# Autodesk Inventor assembly: Intake V3
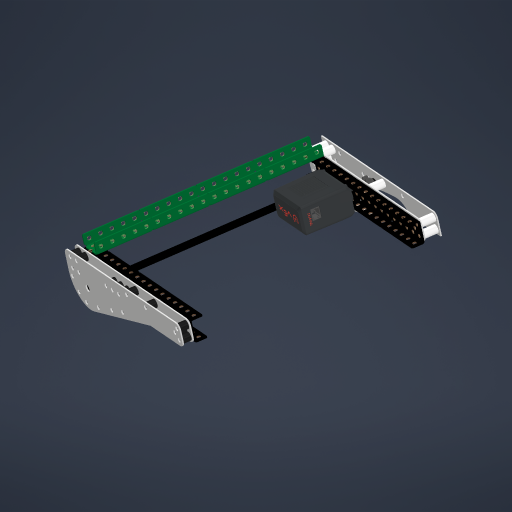
[picture p0: Inventor's stored thumbnail of the model, 512x512]
Saved by Autodesk Inventor 2023.4 (Build 274418000, 418)
## iProperties
Created: 2023-12-16
Part Number: Intake V3
Document SubType Name: Assembly
Designer: diego
Author: diego
## Documents named in this file (20)
- C:\Users\diego\OneDrive\Documents\GitHub\2024-599Z\2024-599Z\Cad\NEW Intake\plan x intake.iam
- C:\Users\diego\OneDrive\Documents\GitHub\2024-599Z\2024-599Z\Cad\Library\VEX-CAD-Inventor-1.4.0\Structure\C Channel\Aluminum 1x2x1\Alu C 1x2x1x17.ipt
- C:\Users\diego\OneDrive\Documents\GitHub\2024-599Z\2024-599Z\Cad\Library\VEX-CAD-Inventor-1.4.0\Motion\Shaft HS\HS Spacer\HSpacer .0625.ipt
- C:\Users\diego\OneDrive\Documents\GitHub\2024-599Z\2024-599Z\Cad\Library\VEX-CAD-Inventor-1.4.0\Motion\Shaft HS\Shaft HS\Shaft HS 11.0 in.ipt
- C:\Users\diego\OneDrive\Documents\GitHub\2024-599Z\2024-599Z\Cad\Library\VEX-CAD-Inventor-1.4.0\Motion\Sprockets\6P Sprocket\6P 8T Sprocket, No Insert.iam
- C:\Users\diego\OneDrive\Documents\GitHub\2024-599Z\2024-599Z\Cad\Library\VEX-CAD-Inventor-1.4.0\Motion\Shaft HS\Low Profile HS Shaft Collar.ipt
- C:\Users\diego\OneDrive\Documents\GitHub\2024-599Z\2024-599Z\Cad\Library\VEX-CAD-Inventor-1.4.0\Motion\Spacers\Spacer Nylon .313 OD\NSpacer .313 OD x .500.ipt
- C:\Users\Meer\OneDrive\Documents\GitHub\2024-599Z\Cad\Library\VEX-CAD-Inventor-1.4.0\Motion\Spacers\Spacer Nylon .313 OD.ipt
- C:\Users\diego\OneDrive\Documents\GitHub\2024-599Z\2024-599Z\Cad\Library\VEX-CAD-Inventor-1.4.0\Motion\Spacers\Spacer Nylon .313 OD\NSpacer .313 OD x .125.ipt
- C:\Users\Meer\OneDrive\Documents\GitHub\2024-599Z\Cad\Library\VEX-CAD-Inventor-1.4.0\Motion\Sprockets\6P Sprocket.iam
- C:\Users\Meer\OneDrive\Documents\GitHub\2024-599Z\Cad\Library\VEX-CAD-Inventor-1.4.0\Motion\Shaft HS\HS Spacer.ipt
- C:\Users\diego\OneDrive\Documents\GitHub\2024-599Z\2024-599Z\Cad\Library\VEX-CAD-Inventor-1.4.0\Motion\Sprockets\6P Sprocket\6P 8T Sprocket, Square.iam
- C:\Users\diego\OneDrive\Documents\GitHub\2024-599Z\2024-599Z\Cad\Library\VEX-CAD-Inventor-1.4.0\Structure\C Channel\Aluminum 1x2x1\Alu C 1x2x1x20.ipt
- C:\Users\Meer\OneDrive\Documents\GitHub\2024-599Z\Cad\Library\VEX-CAD-Inventor-1.4.0\Motion\Shaft HS\Shaft HS.ipt
- C:\Users\diego\OneDrive\Documents\GitHub\2024-599Z\2024-599Z\Cad\NEW CNC Poly\intake poly x.ipt
- C:\Users\diego\OneDrive\Documents\GitHub\2024-599Z\2024-599Z\Cad\Library\VEX-CAD-Inventor-1.4.0\Electronics\Motors with Screws\SteelM-StarS.iam
- C:\Users\Meer\OneDrive\Documents\GitHub\2024-599Z\Cad\Library\VEX-CAD-Inventor-1.4.0\Electronics\Motors with Screws.iam
- C:\Users\diego\OneDrive\Documents\GitHub\2024-599Z\2024-599Z\Cad\Poly for Evan\Intake poly cut (1)\Intake poly cut (1).ipt
- C:\Users\diego\OneDrive\Documents\GitHub\2024-599Z\2024-599Z\Cad\Library\VEX-CAD-Inventor-1.4.0\Motion\Spacers\Spacer Nylon .375 OD\NSpacer .375 OD x .375.ipt
- C:\Users\diego\OneDrive\Documents\GitHub\2024-599Z\2024-599Z\Cad\Library\VEX-CAD-Inventor-1.4.0\Motion\Spacers\Spacer Nylon .375 OD.ipt
## Components (56 placed, 13 different names)
1. Shaft HS 11.0 in:1 — Insert:227
2. Alu C 1x2x1x17:1 — Insert:138, Insert:139, Insert:146, Insert:147, Insert:208, Insert:209
3. Alu C 1x2x1x17:2 — Insert:136, Insert:137, Insert:205, Insert:206, Insert:222
4. 6P 8T Sprocket, No Insert:4 [sub-assembly] — Insert:24, Insert:39
5. HSpacer .0625:8 — Insert:24, Insert:224
6. HSpacer .0625:12 — Insert:39, Insert:225
7. NSpacer .313 OD x .500:1 — Insert:71, Insert:160
8. NSpacer .313 OD x .500:4 — Insert:72, Insert:159
9. NSpacer .313 OD x .500:6 — Insert:63, Insert:150
10. NSpacer .313 OD x .500:8 — Insert:74, Insert:157
11. NSpacer .313 OD x .500:9 — Insert:62, Insert:212
12. NSpacer .313 OD x .500:10 — Insert:61, Insert:214
13. NSpacer .313 OD x .500:12 — Insert:67, Insert:154
14. NSpacer .313 OD x .500:13 — Insert:73, Insert:158
15. NSpacer .313 OD x .500:15 — Insert:69, Insert:156
16. NSpacer .313 OD x .125:19 — Insert:61, Insert:211
17. NSpacer .313 OD x .125:20 — Insert:63
18. NSpacer .313 OD x .125:23 — Insert:62
19. NSpacer .313 OD x .125:24 — Insert:67
20. NSpacer .313 OD x .125:26 — Insert:69, Insert:213
21. NSpacer .313 OD x .125:27 — Insert:71
22. NSpacer .313 OD x .125:29 — Insert:72
23. NSpacer .313 OD x .125:30 — Insert:73
24. NSpacer .313 OD x .125:31 — Insert:74
25. NSpacer .313 OD x .500:34 — Insert:163
26. NSpacer .313 OD x .500:35 — Insert:162
27. NSpacer .313 OD x .125:47
28. NSpacer .313 OD x .125:59
29. Low Profile HS Shaft Collar:4 — Insert:223
30. HSpacer .0625:14 — Insert:135
31. HSpacer .0625:15 — Insert:134, Insert:210
32. 6P 8T Sprocket, Square:6 [sub-assembly] — Insert:134, Insert:135
33. Alu C 1x2x1x20:1 — Insert:136, Insert:137, Insert:138, Insert:139
34. intake poly x:1 — Insert:146, Insert:147, Insert:150, Insert:154, Insert:156, Insert:157, Insert:158, Insert:159, Insert:160, Insert:162, Insert:163, Insert:210, Insert:212, Insert:214, Insert:225
35. intake poly x:2 — Insert:205, Insert:206, Insert:221
36. NSpacer .375 OD x .375:12
37. NSpacer .375 OD x .375:18
38. NSpacer .375 OD x .375:4 — Insert:218
39. NSpacer .375 OD x .375:13
40. NSpacer .375 OD x .375:7 — Insert:219
41. NSpacer .375 OD x .375:5
42. NSpacer .375 OD x .375:3 — Insert:215
43. NSpacer .375 OD x .375:15
44. NSpacer .375 OD x .375:2
45. NSpacer .375 OD x .375:1 — Insert:222, Insert:226
46. NSpacer .375 OD x .375:6 — Insert:216
47. NSpacer .375 OD x .375:10
48. NSpacer .375 OD x .375:14
49. NSpacer .375 OD x .375:16
50. NSpacer .375 OD x .375:11 — Insert:221
51. NSpacer .375 OD x .375:17
52. NSpacer .375 OD x .375:9
53. NSpacer .375 OD x .375:8 — Insert:220
54. intake poly x:3 — Insert:215, Insert:216, Insert:218, Insert:219, Insert:220, Insert:226, Insert:227
55. SteelM-StarS:1 [sub-assembly] — Insert:208, Insert:209
56. Intake poly cut (1):1 — Insert:211, Insert:213, Insert:223, Insert:224
## Relationships (63: Insert 63)
- Insert:24: 6P 8T Sprocket, No Insert:4 ↔ HSpacer .0625:8
- Insert:39: 6P 8T Sprocket, No Insert:4 ↔ HSpacer .0625:12
- Insert:61: NSpacer .313 OD x .500:10 ↔ NSpacer .313 OD x .125:19
- Insert:62: NSpacer .313 OD x .500:9 ↔ NSpacer .313 OD x .125:23
- Insert:63: NSpacer .313 OD x .500:6 ↔ NSpacer .313 OD x .125:20
- Insert:67: NSpacer .313 OD x .500:12 ↔ NSpacer .313 OD x .125:24
- Insert:69: NSpacer .313 OD x .500:15 ↔ NSpacer .313 OD x .125:26
- Insert:71: NSpacer .313 OD x .500:1 ↔ NSpacer .313 OD x .125:27
- Insert:72: NSpacer .313 OD x .500:4 ↔ NSpacer .313 OD x .125:29
- Insert:73: NSpacer .313 OD x .500:13 ↔ NSpacer .313 OD x .125:30
- Insert:74: NSpacer .313 OD x .500:8 ↔ NSpacer .313 OD x .125:31
- [Insert]: NSpacer .313 OD x .500:34 ↔ NSpacer .313 OD x .125:47
- [Insert]: NSpacer .313 OD x .500:35 ↔ NSpacer .313 OD x .125:59
- Insert:134: HSpacer .0625:15 ↔ 6P 8T Sprocket, Square:6
- Insert:135: HSpacer .0625:14 ↔ 6P 8T Sprocket, Square:6
- Insert:136: Alu C 1x2x1x17:2 ↔ Alu C 1x2x1x20:1
- Insert:137: Alu C 1x2x1x17:2 ↔ Alu C 1x2x1x20:1
- Insert:138: Alu C 1x2x1x17:1 ↔ Alu C 1x2x1x20:1
- Insert:139: Alu C 1x2x1x17:1 ↔ Alu C 1x2x1x20:1
- Insert:146: Alu C 1x2x1x17:1 ↔ intake poly x:1
- Insert:147: Alu C 1x2x1x17:1 ↔ intake poly x:1
- Insert:150: NSpacer .313 OD x .500:6 ↔ intake poly x:1
- Insert:154: NSpacer .313 OD x .500:12 ↔ intake poly x:1
- Insert:156: NSpacer .313 OD x .500:15 ↔ intake poly x:1
- Insert:157: NSpacer .313 OD x .500:8 ↔ intake poly x:1
- Insert:158: NSpacer .313 OD x .500:13 ↔ intake poly x:1
- Insert:159: NSpacer .313 OD x .500:4 ↔ intake poly x:1
- Insert:160: NSpacer .313 OD x .500:1 ↔ intake poly x:1
- Insert:162: NSpacer .313 OD x .500:35 ↔ intake poly x:1
- Insert:163: NSpacer .313 OD x .500:34 ↔ intake poly x:1
- [Insert]: NSpacer .375 OD x .375:5 ↔ intake poly x:3
- [Insert]: NSpacer .375 OD x .375:10 ↔ intake poly x:3
- [Insert]: NSpacer .375 OD x .375:16 ↔ intake poly x:3
- [Insert]: NSpacer .375 OD x .375:11 ↔ intake poly x:3
- [Insert]: NSpacer .375 OD x .375:15 ↔ intake poly x:3
- [Insert]: NSpacer .375 OD x .375:14 ↔ intake poly x:3
- [Insert]: NSpacer .375 OD x .375:13 ↔ intake poly x:3
- [Insert]: NSpacer .375 OD x .375:12 ↔ intake poly x:3
- [Insert]: NSpacer .375 OD x .375:18 ↔ intake poly x:3
- [Insert]: NSpacer .375 OD x .375:9 ↔ intake poly x:3
- [Insert]: NSpacer .375 OD x .375:17 ↔ intake poly x:3
- [Insert]: NSpacer .375 OD x .375:2 ↔ intake poly x:3
- Insert:205: Alu C 1x2x1x17:2 ↔ intake poly x:2
- Insert:206: Alu C 1x2x1x17:2 ↔ intake poly x:2
- Insert:208: Alu C 1x2x1x17:1 ↔ SteelM-StarS:1
- Insert:209: Alu C 1x2x1x17:1 ↔ SteelM-StarS:1
- Insert:210: HSpacer .0625:15 ↔ intake poly x:1
- Insert:211: NSpacer .313 OD x .125:19 ↔ Intake poly cut (1):1
- Insert:212: NSpacer .313 OD x .500:9 ↔ intake poly x:1
- Insert:213: NSpacer .313 OD x .125:26 ↔ Intake poly cut (1):1
- Insert:214: NSpacer .313 OD x .500:10 ↔ intake poly x:1
- Insert:215: NSpacer .375 OD x .375:3 ↔ intake poly x:3
- Insert:216: NSpacer .375 OD x .375:6 ↔ intake poly x:3
- Insert:218: NSpacer .375 OD x .375:4 ↔ intake poly x:3
- Insert:219: NSpacer .375 OD x .375:7 ↔ intake poly x:3
- Insert:220: NSpacer .375 OD x .375:8 ↔ intake poly x:3
- Insert:221: intake poly x:2 ↔ NSpacer .375 OD x .375:11
- Insert:222: Alu C 1x2x1x17:2 ↔ NSpacer .375 OD x .375:1
- Insert:223: Low Profile HS Shaft Collar:4 ↔ Intake poly cut (1):1
- Insert:224: HSpacer .0625:8 ↔ Intake poly cut (1):1
- Insert:225: HSpacer .0625:12 ↔ intake poly x:1
- Insert:226: NSpacer .375 OD x .375:1 ↔ intake poly x:3
- Insert:227: Shaft HS 11.0 in:1 ↔ intake poly x:3
## Named parameters: d129_d111 = 0 mm, d141_d124 = 0 mm, d232_d216 = 0 mm, d236_d220 = 0 mm, d237_d221 = 0 mm, d238_d222 = 0 mm, d239_d223 = 0 mm, d240_d224 = 0 mm, d241_d225 = 0 mm, d242_d226 = 0 mm, d243_d227 = 0 mm, d244_d228 = 0 mm, d245_d229 = 0 mm
